# Autodesk Inventor assembly: outer_miirrored
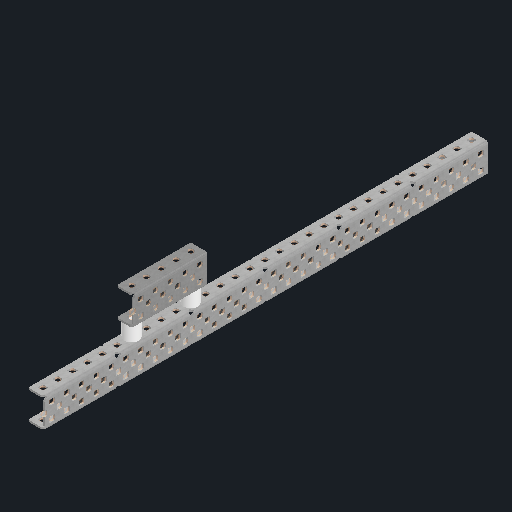
[picture p0: Inventor's stored thumbnail of the model, 512x512]
Saved by Autodesk Inventor 2025 (Build 290162000, 162)
## iProperties
Created: 2024-10-02
Part Number: outer_miirrored
Document SubType Name: Assembly
Designer: Averey Ku
Author: Averey Ku
## Documents named in this file (8)
- D:\vex_robotics_high_stakes\hardware\cad\bots\high_stakes_v2\chassis\drivebay_mirrored\outer_miirrored.iam
- D:\vex_robotics_high_stakes\hardware\cad\bots\high_stakes_v2\chassis\drivebay_mirrored\Alu C 1x2x1x30_miirrored.ipt
- D:\vex_robotics_high_stakes\hardware\cad\bots\high_stakes_v2\chassis\drivebay_mirrored\Bearing Flat Low Profile_miirrored.ipt
- D:\vex_robotics_high_stakes\hardware\cad\robpros_cad_lib\Motion\Spacers\Spacer Nylon .500 OD\NSpacer White .500 OD x .500.ipt
- D:\vex_robotics_high_stakes\hardware\cad\robpros_cad_lib\Motion\Spacers\Spacer Nylon .500 OD.ipt
- D:\vex_robotics_high_stakes\hardware\cad\bots\high_stakes_v2\chassis\drivebay_mirrored\Alu C 1x2x1x5_miirrored.ipt
- D:\vex_robotics_high_stakes\hardware\cad\VEX-CAD-Inventor\Structure\Standoff\Standoff .875.ipt
- D:\vex_robotics_high_stakes\hardware\cad\VEX-CAD-Inventor\Structure\Standoff.ipt
## Components (12 placed, 5 different names)
1. Alu C 1x2x1x30_miirrored:1 — Mate:2, Insert:2, Mate:3, Insert:3, Mate:1, Insert:1, Mate:5, Insert:5, Mate:4, Insert:4, Insert:7, Insert:6, Insert:20, Insert:21
2. Bearing Flat Low Profile_miirrored:1 — Mate:2, Insert:2
3. Bearing Flat Low Profile_miirrored:2 — Mate:3, Insert:3
4. Bearing Flat Low Profile_miirrored:3 — Mate:1, Insert:1
5. Bearing Flat Low Profile_miirrored:4 — Mate:5, Insert:5
6. Bearing Flat Low Profile_miirrored:5 — Mate:4, Insert:4
7. NSpacer White .500 OD x .500:1 — Insert:7, Insert:18
8. NSpacer White .500 OD x .500:2 — Insert:6, Mate:11
9. Bearing Flat Low Profile_miirrored:6 — Mate:12, Insert:19
10. Alu C 1x2x1x5_miirrored:1 — Mate:12, Insert:19, Mate:11, Insert:18
11. Standoff .875:1 — Insert:20
12. Standoff .875:2 — Insert:21
## Relationships (18: Insert 11, Mate 7)
- Mate:2: Alu C 1x2x1x30_miirrored:1 ↔ Bearing Flat Low Profile_miirrored:1
- Insert:2: Alu C 1x2x1x30_miirrored:1 ↔ Bearing Flat Low Profile_miirrored:1
- Mate:3: Alu C 1x2x1x30_miirrored:1 ↔ Bearing Flat Low Profile_miirrored:2
- Insert:3: Alu C 1x2x1x30_miirrored:1 ↔ Bearing Flat Low Profile_miirrored:2
- Mate:1: Alu C 1x2x1x30_miirrored:1 ↔ Bearing Flat Low Profile_miirrored:3
- Insert:1: Alu C 1x2x1x30_miirrored:1 ↔ Bearing Flat Low Profile_miirrored:3
- Mate:5: Alu C 1x2x1x30_miirrored:1 ↔ Bearing Flat Low Profile_miirrored:4
- Insert:5: Alu C 1x2x1x30_miirrored:1 ↔ Bearing Flat Low Profile_miirrored:4
- Mate:4: Alu C 1x2x1x30_miirrored:1 ↔ Bearing Flat Low Profile_miirrored:5
- Insert:4: Alu C 1x2x1x30_miirrored:1 ↔ Bearing Flat Low Profile_miirrored:5
- Insert:7: Alu C 1x2x1x30_miirrored:1 ↔ NSpacer White .500 OD x .500:1
- Insert:6: Alu C 1x2x1x30_miirrored:1 ↔ NSpacer White .500 OD x .500:2
- Mate:12: Bearing Flat Low Profile_miirrored:6 ↔ Alu C 1x2x1x5_miirrored:1
- Insert:19: Bearing Flat Low Profile_miirrored:6 ↔ Alu C 1x2x1x5_miirrored:1
- Mate:11: NSpacer White .500 OD x .500:2 ↔ Alu C 1x2x1x5_miirrored:1
- Insert:18: NSpacer White .500 OD x .500:1 ↔ Alu C 1x2x1x5_miirrored:1
- Insert:20: Alu C 1x2x1x30_miirrored:1 ↔ Standoff .875:1
- Insert:21: Alu C 1x2x1x30_miirrored:1 ↔ Standoff .875:2
